# Autodesk Inventor assembly: 0005-10-01 Cadru
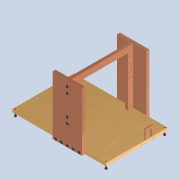
[picture p0: Inventor's stored thumbnail of the model, 180x180]
Saved by Autodesk Inventor 2020 (Build 240168000, 168)
## iProperties
Created: 2020-12-18
Part Number: 0005-10-01 Cadru
Document SubType Name: Assembly
Designer: Iulian Bors
Mass: 17144.8 g
Surface Area: 27601.7 cm^2
Volume: 16303.9 cm^3
Density: 1.05157 g/cm^3
Author: Iulian Bors
Subject: 10-01
## Documents named in this file (8)
- Z:\I.A.B\Proiecte\0005 I.A.B 3d 2.0 Imprimanta aracet\10 Mecanic\0005-10-01 Cadru.iam
- Z:\I.A.B\Proiecte\0005 I.A.B 3d 2.0 Imprimanta aracet\10 Mecanic\0005-10-001-Batiu.ipt
- Z:\I.A.B\Proiecte\0005 I.A.B 3d 2.0 Imprimanta aracet\10 Mecanic\0005-10-017 Batiu 2.ipt
- Z:\I.A.B\Proiecte\0005 I.A.B 3d 2.0 Imprimanta aracet\10 Mecanic\0005-10-024.ipt
- Z:\I.A.B\Proiecte\0005 I.A.B 3d 2.0 Imprimanta aracet\10 Mecanic\0005-10-1022 tiping screw.ipt
- Z:\I.A.B\Proiecte\0005 I.A.B 3d 2.0 Imprimanta aracet\10 Mecanic\0005-10-1023 ISO 4018 - M8 x 40.ipt
- Z:\I.A.B\Proiecte\0005 I.A.B 3d 2.0 Imprimanta aracet\10 Mecanic\0005-10-026 Suport DC in.ipt
- Z:\I.A.B\Proiecte\0005 I.A.B 3d 2.0 Imprimanta aracet\10 Mecanic\0005-10-1027 ISO 7050 - ST 4.2 x 32 - C - Z.ipt
## Components (32 placed, 7 different names)
1. 0005-10-001-Batiu.ipt:1 — Mate:109, Flush:60, Mate:116, Insert:32, Insert:33, Mate:127, Insert:41, Insert:42, Flush:63, Insert:43, Insert:44, Insert:45, Insert:46, Insert:47
2. 0005-10-017 Batiu 2.ipt:2 — Mate:109, Mate:66, Mate:114, Mate:115, Flush:62, Mate:150
3. 0005-10-024.ipt:3 — Flush:60, Mate:114, Mate:115, Flush:61, Insert:28, Mate:126
4. 0005-10-024.ipt:4 — Mate:116, Flush:61, Flush:62, Insert:29, Insert:30
5. 0005-10-1023 ISO 4018 - M8 x 40.ipt:23 — Insert:41
6. 0005-10-1023 ISO 4018 - M8 x 40.ipt:24 — Insert:32
7. 0005-10-1023 ISO 4018 - M8 x 40.ipt:25 — Insert:33
8. 0005-10-1023 ISO 4018 - M8 x 40.ipt:26 — Insert:42
9. 0005-10-026 Suport DC in.ipt:27 — Mate:127, Flush:63
10. 0005-10-1027 ISO 7050 - ST 4.2 x 32 - C - Z.ipt:28 — Insert:43
11. 0005-10-1027 ISO 7050 - ST 4.2 x 32 - C - Z.ipt:29 — Insert:44
12. 0005-10-1022 tiping screw.ipt:30 — Insert:45
13. 0005-10-1022 tiping screw.ipt:31 — Insert:47
14. 0005-10-1022 tiping screw.ipt:32 — Insert:46
15. 0005-10-1022 tiping screw.ipt:5 — Insert:28
16. 0005-10-1022 tiping screw.ipt:6
17. 0005-10-1022 tiping screw.ipt:7
18. 0005-10-1022 tiping screw.ipt:8
19. 0005-10-1022 tiping screw.ipt:9 — Mate:126
20. 0005-10-1022 tiping screw.ipt:10
21. 0005-10-1022 tiping screw.ipt:11
22. 0005-10-1022 tiping screw.ipt:12
23. 0005-10-1022 tiping screw.ipt:13
24. 0005-10-1022 tiping screw.ipt:14 — Insert:29
25. 0005-10-1022 tiping screw.ipt:15
26. 0005-10-1022 tiping screw.ipt:16
27. 0005-10-1022 tiping screw.ipt:17
28. 0005-10-1022 tiping screw.ipt:18 — Insert:30
29. 0005-10-1022 tiping screw.ipt:19
30. 0005-10-1022 tiping screw.ipt:20
31. 0005-10-1022 tiping screw.ipt:21
32. 0005-10-1022 tiping screw.ipt:22
## Component patterns: (4 elements, first: 0005-10-1022 tiping screw.ipt:5), (5 elements, first: 0005-10-1022 tiping screw.ipt:9), (4 elements, first: 0005-10-1022 tiping screw.ipt:14), (5 elements, first: 0005-10-1022 tiping screw.ipt:18)
## Relationships (24: Insert 12, Mate 8, Flush 4)
- Mate:109: 0005-10-001-Batiu.ipt:1 ↔ 0005-10-017 Batiu 2.ipt:2
- Mate:66: 0005-10-017 Batiu 2.ipt:2
- Flush:60: 0005-10-001-Batiu.ipt:1 ↔ 0005-10-024.ipt:3
- Mate:114: 0005-10-017 Batiu 2.ipt:2 ↔ 0005-10-024.ipt:3
- Mate:115: 0005-10-017 Batiu 2.ipt:2 ↔ 0005-10-024.ipt:3
- Mate:116: 0005-10-001-Batiu.ipt:1 ↔ 0005-10-024.ipt:4
- Flush:61: 0005-10-024.ipt:3 ↔ 0005-10-024.ipt:4
- Flush:62: 0005-10-017 Batiu 2.ipt:2 ↔ 0005-10-024.ipt:4
- Insert:28: 0005-10-024.ipt:3 ↔ 0005-10-1022 tiping screw.ipt:5
- Mate:126: 0005-10-024.ipt:3 ↔ 0005-10-1022 tiping screw.ipt:9
- Insert:29: 0005-10-024.ipt:4 ↔ 0005-10-1022 tiping screw.ipt:14
- Insert:30: 0005-10-024.ipt:4 ↔ 0005-10-1022 tiping screw.ipt:18
- Insert:32: 0005-10-001-Batiu.ipt:1 ↔ 0005-10-1023 ISO 4018 - M8 x 40.ipt:24
- Insert:33: 0005-10-001-Batiu.ipt:1 ↔ 0005-10-1023 ISO 4018 - M8 x 40.ipt:25
- Mate:127: 0005-10-001-Batiu.ipt:1 ↔ 0005-10-026 Suport DC in.ipt:27
- Insert:41: 0005-10-001-Batiu.ipt:1 ↔ 0005-10-1023 ISO 4018 - M8 x 40.ipt:23
- Insert:42: 0005-10-001-Batiu.ipt:1 ↔ 0005-10-1023 ISO 4018 - M8 x 40.ipt:26
- Mate:150 (120 mm): 0005-10-017 Batiu 2.ipt:2
- Flush:63: 0005-10-001-Batiu.ipt:1 ↔ 0005-10-026 Suport DC in.ipt:27
- Insert:43: 0005-10-001-Batiu.ipt:1 ↔ 0005-10-1027 ISO 7050 - ST 4.2 x 32 - C - Z.ipt:28
- Insert:44: 0005-10-001-Batiu.ipt:1 ↔ 0005-10-1027 ISO 7050 - ST 4.2 x 32 - C - Z.ipt:29
- Insert:45: 0005-10-001-Batiu.ipt:1 ↔ 0005-10-1022 tiping screw.ipt:30
- Insert:46: 0005-10-001-Batiu.ipt:1 ↔ 0005-10-1022 tiping screw.ipt:32
- Insert:47: 0005-10-001-Batiu.ipt:1 ↔ 0005-10-1022 tiping screw.ipt:31
